# Autodesk Inventor assembly: force_sensor_plate
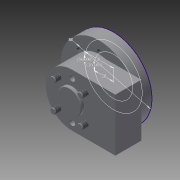
[picture p0: Inventor's stored thumbnail of the model, 180x180]
Saved by Autodesk Inventor 2013 (Build 170138000, 138)
## iProperties
Created: 2013-01-30
Part Number: force_sensor_plate
Document SubType Name: Assembly
Designer: Mahisorn
Author: Mahisorn
## Documents named in this file (4)
- E:\mahisorn\documents\hg-ros-pkg\cad\gripper\force_sensor_plate.iam
- E:\mahisorn\documents\hg-ros-pkg\cad\gripper\CFS055CA501U.ipt
- E:\mahisorn\documents\hg-ros-pkg\cad\gripper\plate_for_CFS055CA501U.ipt
- E:\mahisorn\documents\Inventor\Content Center Files\R2013\en-US\ANSI B18.3.1M(5)\ANSI B18.3.1M - M6x1 x 12(3).ipt
## Components (6 placed, 3 different names)
1. CFS055CA501U:1 — Mate:1
2. plate_for_CFS055CA501U:1 — Mate:1, Insert:1, Insert:2, Insert:3, Insert:4
3. Drilled Forged Hexagon Socket Head Cap Screw - 6 Holes - Metric M6x1 x 12:1 — Insert:3
4. Drilled Forged Hexagon Socket Head Cap Screw - 6 Holes - Metric M6x1 x 12:2 — Insert:4
5. Drilled Forged Hexagon Socket Head Cap Screw - 6 Holes - Metric M6x1 x 12:3 — Insert:2
6. Drilled Forged Hexagon Socket Head Cap Screw - 6 Holes - Metric M6x1 x 12:4 — Insert:1
## Relationships (5: Insert 4, Mate 1)
- Mate:1: CFS055CA501U:1 ↔ plate_for_CFS055CA501U:1
- Insert:1: plate_for_CFS055CA501U:1 ↔ Drilled Forged Hexagon Socket Head Cap Screw - 6 Holes - Metric M6x1 x 12:4
- Insert:2: plate_for_CFS055CA501U:1 ↔ Drilled Forged Hexagon Socket Head Cap Screw - 6 Holes - Metric M6x1 x 12:3
- Insert:3: plate_for_CFS055CA501U:1 ↔ Drilled Forged Hexagon Socket Head Cap Screw - 6 Holes - Metric M6x1 x 12:1
- Insert:4: plate_for_CFS055CA501U:1 ↔ Drilled Forged Hexagon Socket Head Cap Screw - 6 Holes - Metric M6x1 x 12:2
